# Autodesk Inventor assembly: Assembly3
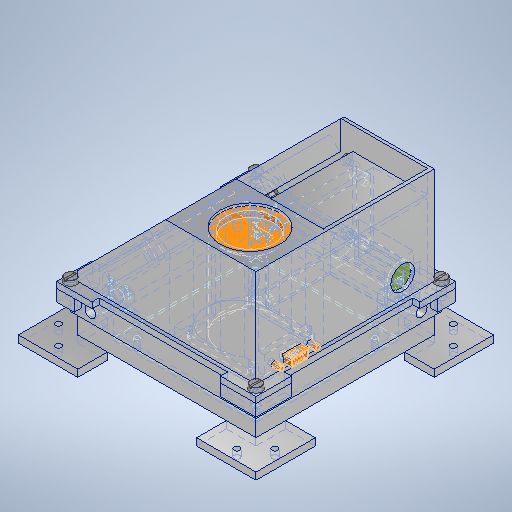
[picture p0: Inventor's stored thumbnail of the model, 512x512]
Saved by Autodesk Inventor 2025 (Build 290162000, 162)
## iProperties
Created: 2024-04-12
Part Number: Assembly3
Document SubType Name: Assembly
Designer: mahal
Author: mahal
## Documents named in this file (4)
- A:\study\IIST  COURSE\4th sem\MACHINING\project\Assembly3.iam
- A:\study\IIST  COURSE\4th sem\MACHINING\project\Assembly1.iam
- A:\study\IIST  COURSE\4th sem\MACHINING\project\Assembly2.iam
- C:\Users\mahal\OneDrive\Documents\Inventor\Content Center Files\R2025\en-US\UNI 6107\UNI 6107 - M6 x  10.ipt
## Components (6 placed, 3 different names)
1. Assembly1:1 [sub-assembly] — Insert:1, Insert:2, Insert:3, Insert:4, Insert:5
2. Assembly2:1 [sub-assembly] — Insert:1
3. UNI 6107 M6 x  10:1 — Insert:2
4. UNI 6107 M6 x  10:2 — Insert:3
5. UNI 6107 M6 x  10:3 — Insert:4
6. UNI 6107 M6 x  10:4 — Insert:5
## Relationships (5: Insert 5)
- Insert:1: Assembly1:1 ↔ Assembly2:1
- Insert:2: Assembly1:1 ↔ UNI 6107 M6 x  10:1
- Insert:3: Assembly1:1 ↔ UNI 6107 M6 x  10:2
- Insert:4: Assembly1:1 ↔ UNI 6107 M6 x  10:3
- Insert:5: Assembly1:1 ↔ UNI 6107 M6 x  10:4
